# Autodesk Inventor assembly: platform
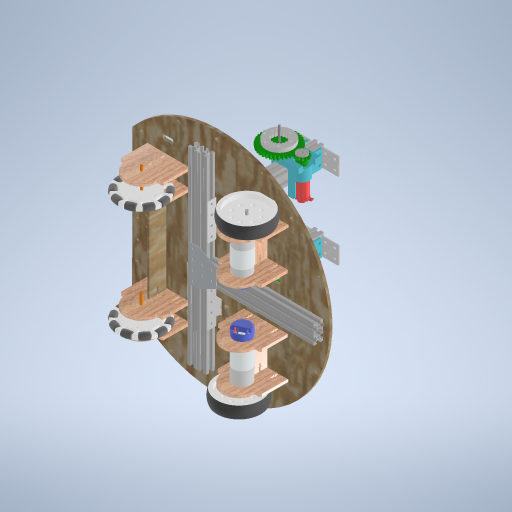
[picture p0: Inventor's stored thumbnail of the model, 512x512]
Saved by Autodesk Inventor 2024 (Build 280153000, 153)
## iProperties
Created: 2023-03-13
Part Number: platform
Document SubType Name: Assembly
Designer: User
Author: User
## Documents named in this file (42)
- C:\Users\ejenie\reposGits\Cheburashka\Cheburashka_construction\platform\platform.iam
- C:\Users\ejenie\reposGits\Cheburashka\Cheburashka_construction\platform\Osn. platform.ipt
- C:\Users\ejenie\reposGits\Cheburashka\Cheburashka_construction\platform\motor1.ipt
- C:\Users\ejenie\reposGits\Cheburashka\Cheburashka_construction\platform\motor2.ipt
- C:\Users\ejenie\reposGits\Cheburashka\Cheburashka_construction\platform\motor3.ipt
- C:\Users\ejenie\reposGits\Cheburashka\Cheburashka_construction\platform\wheel1.ipt
- C:\Users\ejenie\reposGits\Cheburashka\Cheburashka_construction\platform\44260_txm torquenado dc motor_MIR2.ipt
- C:\Users\ejenie\reposGits\Cheburashka\Cheburashka_construction\platform\36466_txm-4 inch omni wheel.ipt
- C:\Users\ejenie\reposGits\Cheburashka\Cheburashka_construction\platform\39055_txm-4 inch wheel_MIR1.ipt
- C:\Users\ejenie\reposGits\Cheburashka\Cheburashka_construction\platform\motor1_MIR3.ipt
- C:\Users\ejenie\reposGits\Cheburashka\Cheburashka_construction\platform\motor2_MIR3.ipt
- C:\Users\ejenie\reposGits\Cheburashka\Cheburashka_construction\platform\motor3_MIR3.ipt
- C:\Users\ejenie\reposGits\Cheburashka\Cheburashka_construction\platform\44260_txm torquenado dc motor_MIR2_MIR.ipt
- C:\Users\ejenie\reposGits\Cheburashka\Cheburashka_construction\platform\wheel1_MIR.ipt
- C:\Users\ejenie\reposGits\Cheburashka\Cheburashka_construction\platform\36466_txm-4 inch omni wheel_MIR2.ipt
- C:\Users\ejenie\reposGits\Cheburashka\Cheburashka_construction\platform\39055_txm-4 inch wheel_MIR1_MIR.ipt
- C:\Users\ejenie\reposGits\Cheburashka\Cheburashka_construction\platform\ось колес2.ipt
- C:\Users\ejenie\reposGits\Cheburashka\Cheburashka_construction\platform\обр_профиль.ipt
- C:\Users\ejenie\reposGits\Cheburashka\Cheburashka_construction\platform\обр_профиль2.ipt
- C:\Users\ejenie\reposGits\Cheburashka\Cheburashka_construction\platform\8bc17c1464c21f56fb2a3979b7c6b729.ipt
- C:\Users\ejenie\reposGits\Cheburashka\Cheburashka_construction\platform\L72-T_soedinitel-60kh80.ipt
- C:\Users\ejenie\reposGits\Cheburashka\Cheburashka_construction\platform\ребро.ipt
- C:\Users\ejenie\reposGits\Cheburashka\Cheburashka_construction\platform\4ad8d019baf454c6bbd45c2c6ffb6783.ipt
- C:\Users\ejenie\reposGits\Cheburashka\Cheburashka_construction\platform\legs\myMotorHolder.ipt
- C:\Users\ejenie\reposGits\Cheburashka\Cheburashka_construction\platform\legs\POLULU final.ipt
- C:\Users\ejenie\reposGits\Cheburashka\Cheburashka_construction\platform\legs\axis.ipt
- C:\Users\ejenie\reposGits\Cheburashka\Cheburashka_construction\platform\legs\bering.ipt
- C:\Users\ejenie\reposGits\Cheburashka\Cheburashka_construction\platform\8bc17c1464c21f56fb2a3979b7c6b729_MIR.ipt
- C:\Users\ejenie\reposGits\Cheburashka\Cheburashka_construction\platform\8bc17c1464c21f56fb2a3979b7c6b729_MIR1.ipt
- C:\Users\ejenie\reposGits\Cheburashka\Cheburashka_construction\platform\подш_ноги.ipt
- C:\Users\ejenie\reposGits\Cheburashka\Cheburashka_construction\platform\legs\шестерня12_туу.ipt
- C:\Users\ejenie\reposGits\Cheburashka\Cheburashka_construction\platform\legs\шестерня36_туу.ipt
- C:\Users\ejenie\reposGits\Cheburashka\Cheburashka_construction\korpus\цил1.ipt
- C:\Users\ejenie\Downloads\Фланец_5мм\Фланец_5мм.ipt
- C:\Users\ejenie\reposGits\Cheburashka\Cheburashka_construction\platform\legs\myMotorHolder_MIR1.ipt
- C:\Users\ejenie\reposGits\Cheburashka\Cheburashka_construction\platform\legs\POLULU final_MIR1.ipt
- C:\Users\ejenie\reposGits\Cheburashka\Cheburashka_construction\platform\legs\axis_MIR1.ipt
- C:\Users\ejenie\reposGits\Cheburashka\Cheburashka_construction\platform\legs\bering_MIR1.ipt
- C:\Users\ejenie\reposGits\Cheburashka\Cheburashka_construction\platform\legs\шестерня12_туу_MIR1.ipt
- C:\Users\ejenie\reposGits\Cheburashka\Cheburashka_construction\platform\legs\шестерня36_туу_MIR.ipt
- C:\Users\ejenie\reposGits\Cheburashka\Cheburashka_construction\korpus\цил1_MIR1.ipt
- C:\Users\ejenie\Downloads\Фланец_5мм\Фланец_5мм_MIR1.ipt
## Components (51 placed, 41 different names)
1. Osn. platform:1 — Совмещение:129, Совмещение:130, Совмещение:131, Совмещение:132, Совмещение:133, Совмещение:137, Совмещение:138, Совмещение:155, Совмещение:158, Совмещение:178, Совмещение:181, Совмещение:182, Совмещение:183, Совмещение:184, Совмещение:185, Совмещение:186, Совмещение:192, Совмещение:193, Совмещение:194, Совмещение:195, Совмещение:196, Совмещение:197, Совмещение:198, Совмещение:230, Совмещение:231, Совмещение:232, Совмещение:233, Совмещение:280, Совмещение:281, Совмещение:282, Совмещение:302, Совмещение:303, Совмещение:304, Совмещение:305
2. motor1:1 — Совмещение:181, Совмещение:182
3. motor2:1 — Совмещение:232, Совмещение:233, Совмещение:306
4. motor3:1 — Совмещение:230, Совмещение:231, Совмещение:307
5. 44260_txm torquenado dc motor_MIR2:1 — Совмещение:21, Совмещение:306, Совмещение:307
6. myMotorHolder:1 — Совмещение:247, Заподлицо:4, Совмещение:289, Совмещение:290, Совмещение:291, Совмещение:292, Совмещение:293, Совмещение:295, Совмещение:296, Совмещение:298, Совмещение:314
7. wheel1:1 — Совмещение:185, Совмещение:186
8. 36466_txm-4 inch omni wheel:1 — Совмещение:308
9. 39055_txm-4 inch wheel_MIR1:1 — Совмещение:21
10. motor1_MIR3:1 — Совмещение:183, Совмещение:184
11. motor2_MIR3:1 — Совмещение:148, Совмещение:304, Совмещение:305
12. motor3_MIR3:1 — Совмещение:110, Совмещение:111, Совмещение:302, Совмещение:303
13. 44260_txm torquenado dc motor_MIR2_MIR:1 — Совмещение:110, Совмещение:148
14. wheel1_MIR:1 — Совмещение:192, Совмещение:197, Совмещение:198, Совмещение:228
15. wheel1_MIR:2 — Совмещение:195, Совмещение:196
16. 36466_txm-4 inch omni wheel_MIR2:1 — Совмещение:229
17. 39055_txm-4 inch wheel_MIR1_MIR:1 — Совмещение:111
18. ось колес2:1 — Совмещение:228, Совмещение:229, Совмещение:308
19. обр_профиль:1 — Совмещение:129, Совмещение:130, Совмещение:131, Совмещение:179, Совмещение:206, Совмещение:207, Совмещение:208, Совмещение:210, Симметрия:1, Совмещение:331, Заподлицо:7, Заподлицо:8, Совмещение:352
20. обр_профиль:2 — Совмещение:132, Совмещение:133, Совмещение:135, Совмещение:136, Совмещение:157, Совмещение:212, Совмещение:237, Совмещение:238, Совмещение:242, Совмещение:243, Заподлицо:1, Заподлицо:2, Симметрия:1, Совмещение:290
21. обр_профиль2:1 — Совмещение:135, Совмещение:136, Совмещение:139, Совмещение:204, Совмещение:205, Совмещение:209, Совмещение:211
22. обр_профиль:3 — Совмещение:137, Совмещение:138, Совмещение:139
23. 8bc17c1464c21f56fb2a3979b7c6b729:1 — Совмещение:155, Совмещение:206, Совмещение:207
24. 8bc17c1464c21f56fb2a3979b7c6b729:2 — Совмещение:157, Совмещение:158
25. L72-T_soedinitel-60kh80:1 — Совмещение:209, Совмещение:210
26. L72-T_soedinitel-60kh80:2 — Совмещение:211, Совмещение:212
27. L72-T_soedinitel-60kh80:3 — Совмещение:204, Совмещение:205
28. ребро:1 — Совмещение:201, Совмещение:202, Совмещение:203
29. 4ad8d019baf454c6bbd45c2c6ffb6783:1 — Совмещение:178, Совмещение:179, Совмещение:208
30. wheel1:2 — Совмещение:193, Совмещение:194, Совмещение:201, Совмещение:202, Совмещение:203
31. 8bc17c1464c21f56fb2a3979b7c6b729:3 — Совмещение:237, Совмещение:238, Заподлицо:2, Совмещение:291, Заподлицо:10
32. 8bc17c1464c21f56fb2a3979b7c6b729:4 — Совмещение:242, Совмещение:243, Заподлицо:1, Совмещение:292
33. POLULU final:1 — Совмещение:247, Совмещение:295, Совмещение:319
34. axis:1 — Совмещение:301
35. bering:1 — Совмещение:289, Совмещение:293
36. 8bc17c1464c21f56fb2a3979b7c6b729_MIR:1 — Заподлицо:6, Совмещение:349, Заподлицо:7, Совмещение:351, Заподлицо:9, Совмещение:352, Совмещение:353, Заподлицо:10
37. 4ad8d019baf454c6bbd45c2c6ffb6783:2 — Совмещение:280, Совмещение:281, Совмещение:282
38. 8bc17c1464c21f56fb2a3979b7c6b729_MIR1:1 — Заподлицо:6, Совмещение:331, Заподлицо:8, Заподлицо:9
39. подш_ноги:1 — Заподлицо:4, Совмещение:297, Совмещение:298
40. шестерня12_туу:1 — Совмещение:314, Совмещение:315, Совмещение:316, Совмещение:317, Совмещение:318
41. шестерня36_туу:1 — Совмещение:296, Совмещение:297, Совмещение:301, Заподлицо:5, Совмещение:309, Совмещение:310
42. цил1:1 — Заподлицо:5, Совмещение:309, Совмещение:310
43. Фланец_5мм:1 — Совмещение:315, Совмещение:316, Совмещение:317, Совмещение:318, Совмещение:319
44. myMotorHolder_MIR1:1 — Совмещение:332, Совмещение:333, Совмещение:334, Совмещение:335, Совмещение:336, Совмещение:338, Совмещение:348, Совмещение:349, Совмещение:351, Совмещение:353
45. POLULU final_MIR1:1 — Совмещение:332, Совмещение:333, Совмещение:342
46. axis_MIR1:1 — Совмещение:337
47. bering_MIR1:1 — Совмещение:334, Совмещение:335
48. шестерня12_туу_MIR1:1 — Совмещение:336, Совмещение:343, Совмещение:344, Совмещение:345, Совмещение:346
49. шестерня36_туу_MIR:1 — Совмещение:337, Совмещение:338, Совмещение:339, Совмещение:340, Совмещение:341, Совмещение:348
50. цил1_MIR1:1 — Совмещение:339, Совмещение:340, Совмещение:341
51. Фланец_5мм_MIR1:1 — Совмещение:342, Совмещение:343, Совмещение:344, Совмещение:345, Совмещение:346
## Relationships (114: Mate 104, Flush 9, Symmetry 1)
- Совмещение:21 [Mate]: 44260_txm torquenado dc motor_MIR2:1 ↔ 39055_txm-4 inch wheel_MIR1:1
- Совмещение:110 [Mate]: motor3_MIR3:1 ↔ 44260_txm torquenado dc motor_MIR2_MIR:1
- Совмещение:111 [Mate] (5 mm): motor3_MIR3:1 ↔ 39055_txm-4 inch wheel_MIR1_MIR:1
- Совмещение:129 [Mate]: Osn. platform:1 ↔ обр_профиль:1
- Совмещение:130 [Mate]: Osn. platform:1 ↔ обр_профиль:1
- Совмещение:131 [Mate]: Osn. platform:1 ↔ обр_профиль:1
- Совмещение:132 [Mate]: Osn. platform:1 ↔ обр_профиль:2
- Совмещение:133 [Mate]: Osn. platform:1 ↔ обр_профиль:2
- Совмещение:135 [Mate] (99.253 mm): обр_профиль:2 ↔ обр_профиль2:1
- Совмещение:136 [Mate]: обр_профиль:2 ↔ обр_профиль2:1
- Совмещение:137 [Mate]: Osn. platform:1 ↔ обр_профиль:3
- Совмещение:138 [Mate] (4.43 mm): Osn. platform:1 ↔ обр_профиль:3
- Совмещение:139 [Mate]: обр_профиль2:1 ↔ обр_профиль:3
- Совмещение:148 [Mate]: motor2_MIR3:1 ↔ 44260_txm torquenado dc motor_MIR2_MIR:1
- Совмещение:155 [Mate]: Osn. platform:1 ↔ 8bc17c1464c21f56fb2a3979b7c6b729:1
- Совмещение:157 [Mate]: обр_профиль:2 ↔ 8bc17c1464c21f56fb2a3979b7c6b729:2
- Совмещение:158 [Mate]: Osn. platform:1 ↔ 8bc17c1464c21f56fb2a3979b7c6b729:2
- Совмещение:178 [Mate]: Osn. platform:1 ↔ 4ad8d019baf454c6bbd45c2c6ffb6783:1
- Совмещение:179 [Mate]: обр_профиль:1 ↔ 4ad8d019baf454c6bbd45c2c6ffb6783:1
- Совмещение:181 [Mate]: Osn. platform:1 ↔ motor1:1
- Совмещение:182 [Mate]: Osn. platform:1 ↔ motor1:1
- Совмещение:183 [Mate]: Osn. platform:1 ↔ motor1_MIR3:1
- Совмещение:184 [Mate]: Osn. platform:1 ↔ motor1_MIR3:1
- Совмещение:185 [Mate]: Osn. platform:1 ↔ wheel1:1
- Совмещение:186 [Mate]: Osn. platform:1 ↔ wheel1:1
- Совмещение:192 [Mate]: Osn. platform:1 ↔ wheel1_MIR:1
- Совмещение:193 [Mate]: Osn. platform:1 ↔ wheel1:2
- Совмещение:194 [Mate]: Osn. platform:1 ↔ wheel1:2
- Совмещение:195 [Mate]: Osn. platform:1 ↔ wheel1_MIR:2
- Совмещение:196 [Mate]: Osn. platform:1 ↔ wheel1_MIR:2
- Совмещение:197 [Mate]: Osn. platform:1 ↔ wheel1_MIR:1
- Совмещение:198 [Mate]: Osn. platform:1 ↔ wheel1_MIR:1
- Совмещение:201 [Mate]: ребро:1 ↔ wheel1:2
- Совмещение:202 [Mate]: ребро:1 ↔ wheel1:2
- Совмещение:203 [Mate]: ребро:1 ↔ wheel1:2
- Совмещение:204 [Mate]: обр_профиль2:1 ↔ L72-T_soedinitel-60kh80:3
- Совмещение:205 [Mate]: обр_профиль2:1 ↔ L72-T_soedinitel-60kh80:3
- Совмещение:206 [Mate]: обр_профиль:1 ↔ 8bc17c1464c21f56fb2a3979b7c6b729:1
- Совмещение:207 [Mate]: обр_профиль:1 ↔ 8bc17c1464c21f56fb2a3979b7c6b729:1
- Совмещение:208 [Mate]: обр_профиль:1 ↔ 4ad8d019baf454c6bbd45c2c6ffb6783:1
- Совмещение:209 [Mate]: обр_профиль2:1 ↔ L72-T_soedinitel-60kh80:1
- Совмещение:210 [Mate]: обр_профиль:1 ↔ L72-T_soedinitel-60kh80:1
- Совмещение:211 [Mate]: обр_профиль2:1 ↔ L72-T_soedinitel-60kh80:2
- Совмещение:212 [Mate]: обр_профиль:2 ↔ L72-T_soedinitel-60kh80:2
- Совмещение:228 [Mate]: wheel1_MIR:1 ↔ ось колес2:1
- Совмещение:229 [Mate]: 36466_txm-4 inch omni wheel_MIR2:1 ↔ ось колес2:1
- Совмещение:230 [Mate]: Osn. platform:1 ↔ motor3:1
- Совмещение:231 [Mate]: Osn. platform:1 ↔ motor3:1
- Совмещение:232 [Mate]: Osn. platform:1 ↔ motor2:1
- Совмещение:233 [Mate]: Osn. platform:1 ↔ motor2:1
- Совмещение:237 [Mate]: обр_профиль:2 ↔ 8bc17c1464c21f56fb2a3979b7c6b729:3
- Совмещение:238 [Mate]: обр_профиль:2 ↔ 8bc17c1464c21f56fb2a3979b7c6b729:3
- Совмещение:242 [Mate]: обр_профиль:2 ↔ 8bc17c1464c21f56fb2a3979b7c6b729:4
- Совмещение:243 [Mate]: обр_профиль:2 ↔ 8bc17c1464c21f56fb2a3979b7c6b729:4
- Совмещение:247 [Mate]: myMotorHolder:1 ↔ POLULU final:1
- Заподлицо:1 [Flush] (4 mm): обр_профиль:2 ↔ 8bc17c1464c21f56fb2a3979b7c6b729:4
- Заподлицо:2 [Flush] (4 mm): обр_профиль:2 ↔ 8bc17c1464c21f56fb2a3979b7c6b729:3
- Симметрия:1 [Symmetry]: обр_профиль:1 ↔ обр_профиль:2
- Совмещение:280 [Mate]: Osn. platform:1 ↔ 4ad8d019baf454c6bbd45c2c6ffb6783:2
- Совмещение:281 [Mate]: Osn. platform:1 ↔ 4ad8d019baf454c6bbd45c2c6ffb6783:2
- Совмещение:282 [Mate]: Osn. platform:1 ↔ 4ad8d019baf454c6bbd45c2c6ffb6783:2
- Заподлицо:4 [Flush]: myMotorHolder:1 ↔ подш_ноги:1
- Совмещение:289 [Mate]: myMotorHolder:1 ↔ bering:1
- Совмещение:290 [Mate]: myMotorHolder:1 ↔ обр_профиль:2
- Совмещение:291 [Mate]: myMotorHolder:1 ↔ 8bc17c1464c21f56fb2a3979b7c6b729:3
- Совмещение:292 [Mate]: myMotorHolder:1 ↔ 8bc17c1464c21f56fb2a3979b7c6b729:4
- Совмещение:293 [Mate]: myMotorHolder:1 ↔ bering:1
- Совмещение:295 [Mate]: myMotorHolder:1 ↔ POLULU final:1
- Совмещение:296 [Mate]: myMotorHolder:1 ↔ шестерня36_туу:1
- Совмещение:297 [Mate]: подш_ноги:1 ↔ шестерня36_туу:1
- Совмещение:298 [Mate]: myMotorHolder:1 ↔ подш_ноги:1
- Совмещение:301 [Mate]: axis:1 ↔ шестерня36_туу:1
- Совмещение:302 [Mate]: Osn. platform:1 ↔ motor3_MIR3:1
- Совмещение:303 [Mate]: Osn. platform:1 ↔ motor3_MIR3:1
- Совмещение:304 [Mate]: Osn. platform:1 ↔ motor2_MIR3:1
- Совмещение:305 [Mate]: Osn. platform:1 ↔ motor2_MIR3:1
- Совмещение:306 [Mate]: motor2:1 ↔ 44260_txm torquenado dc motor_MIR2:1
- Совмещение:307 [Mate]: motor3:1 ↔ 44260_txm torquenado dc motor_MIR2:1
- Совмещение:308 [Mate]: 36466_txm-4 inch omni wheel:1 ↔ ось колес2:1
- Заподлицо:5 [Flush]: шестерня36_туу:1 ↔ цил1:1
- Совмещение:309 [Mate]: шестерня36_туу:1 ↔ цил1:1
- Совмещение:310 [Mate]: шестерня36_туу:1 ↔ цил1:1
- Совмещение:314 [Mate]: myMotorHolder:1 ↔ шестерня12_туу:1
- Совмещение:315 [Mate]: шестерня12_туу:1 ↔ Фланец_5мм:1
- Совмещение:316 [Mate]: шестерня12_туу:1 ↔ Фланец_5мм:1
- Совмещение:317 [Mate]: шестерня12_туу:1 ↔ Фланец_5мм:1
- Совмещение:318 [Mate]: шестерня12_туу:1 ↔ Фланец_5мм:1
- Совмещение:319 [Mate]: POLULU final:1 ↔ Фланец_5мм:1
- Заподлицо:6 [Flush]: 8bc17c1464c21f56fb2a3979b7c6b729_MIR:1 ↔ 8bc17c1464c21f56fb2a3979b7c6b729_MIR1:1
- Совмещение:331 [Mate]: обр_профиль:1 ↔ 8bc17c1464c21f56fb2a3979b7c6b729_MIR1:1
- Совмещение:332 [Mate]: myMotorHolder_MIR1:1 ↔ POLULU final_MIR1:1
- Совмещение:333 [Mate]: myMotorHolder_MIR1:1 ↔ POLULU final_MIR1:1
- Совмещение:334 [Mate]: myMotorHolder_MIR1:1 ↔ bering_MIR1:1
- Совмещение:335 [Mate]: myMotorHolder_MIR1:1 ↔ bering_MIR1:1
- Совмещение:336 [Mate]: myMotorHolder_MIR1:1 ↔ шестерня12_туу_MIR1:1
- Совмещение:337 [Mate]: axis_MIR1:1 ↔ шестерня36_туу_MIR:1
- Совмещение:338 [Mate]: myMotorHolder_MIR1:1 ↔ шестерня36_туу_MIR:1
- Совмещение:339 [Mate]: шестерня36_туу_MIR:1 ↔ цил1_MIR1:1
- Совмещение:340 [Mate]: шестерня36_туу_MIR:1 ↔ цил1_MIR1:1
- Совмещение:341 [Mate]: шестерня36_туу_MIR:1 ↔ цил1_MIR1:1
- Совмещение:342 [Mate]: POLULU final_MIR1:1 ↔ Фланец_5мм_MIR1:1
- Совмещение:343 [Mate]: шестерня12_туу_MIR1:1 ↔ Фланец_5мм_MIR1:1
- Совмещение:344 [Mate]: шестерня12_туу_MIR1:1 ↔ Фланец_5мм_MIR1:1
- Совмещение:345 [Mate]: шестерня12_туу_MIR1:1 ↔ Фланец_5мм_MIR1:1
- Совмещение:346 [Mate]: шестерня12_туу_MIR1:1 ↔ Фланец_5мм_MIR1:1
- Совмещение:348 [Mate]: myMotorHolder_MIR1:1 ↔ шестерня36_туу_MIR:1
- Совмещение:349 [Mate]: 8bc17c1464c21f56fb2a3979b7c6b729_MIR:1 ↔ myMotorHolder_MIR1:1
- Заподлицо:7 [Flush]: обр_профиль:1 ↔ 8bc17c1464c21f56fb2a3979b7c6b729_MIR:1
- Заподлицо:8 [Flush]: обр_профиль:1 ↔ 8bc17c1464c21f56fb2a3979b7c6b729_MIR1:1
- Совмещение:351 [Mate]: 8bc17c1464c21f56fb2a3979b7c6b729_MIR:1 ↔ myMotorHolder_MIR1:1
- Заподлицо:9 [Flush]: 8bc17c1464c21f56fb2a3979b7c6b729_MIR:1 ↔ 8bc17c1464c21f56fb2a3979b7c6b729_MIR1:1
- Совмещение:352 [Mate]: обр_профиль:1 ↔ 8bc17c1464c21f56fb2a3979b7c6b729_MIR:1
- Совмещение:353 [Mate]: 8bc17c1464c21f56fb2a3979b7c6b729_MIR:1 ↔ myMotorHolder_MIR1:1
- Заподлицо:10 [Flush]: 8bc17c1464c21f56fb2a3979b7c6b729:3 ↔ 8bc17c1464c21f56fb2a3979b7c6b729_MIR:1
